# Autodesk Inventor assembly: Body
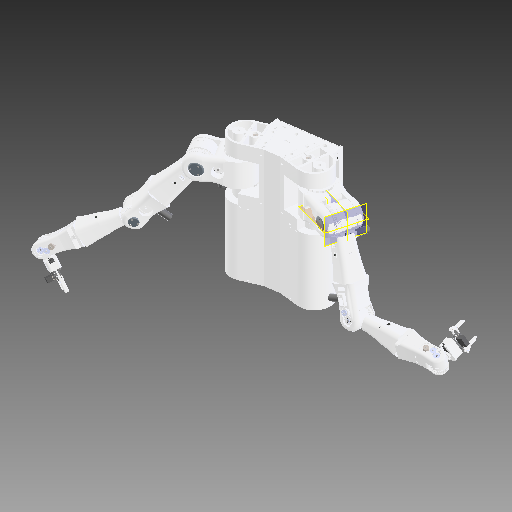
[picture p0: Inventor's stored thumbnail of the model, 512x512]
Saved by Autodesk Inventor 2017 (Build 210142000, 142)
## iProperties
Created: 2017-03-13
Part Number: Body
Document SubType Name: Assembly
Designer: zallen
Author: zallen
## Documents named in this file (4)
- C:\Users\Dell\Documents\GitHub\tr1\src\Body\Body.iam
- C:\Users\Dell\Documents\GitHub\tr1\src\Body\Chest Assembly\Chest Assembly.iam
- C:\Users\Dell\Documents\GitHub\tr1\src\Body\Arm Assembly\Arm Assembly, Right.iam
- C:\Users\Dell\Documents\GitHub\tr1\src\Body\Arm Assembly\Arm Assembly, Left.iam
## Components (3 placed, 3 different names)
1. Chest Assembly:1 [sub-assembly] — Mate:15, Mate:16, Flush:1, Mate:17, Flush:2, Mate:18
2. Arm Assembly, Right:1 [sub-assembly] — Mate:15, Mate:16, Flush:1
3. Arm Assembly, Left:1 [sub-assembly] — Mate:17, Flush:2, Mate:18
## Relationships (6: Mate 4, Flush 2)
- Mate:15: Chest Assembly:1 ↔ Arm Assembly, Right:1
- Mate:16: Chest Assembly:1 ↔ Arm Assembly, Right:1
- Flush:1: Chest Assembly:1 ↔ Arm Assembly, Right:1
- Mate:17: Chest Assembly:1 ↔ Arm Assembly, Left:1
- Flush:2: Chest Assembly:1 ↔ Arm Assembly, Left:1
- Mate:18: Chest Assembly:1 ↔ Arm Assembly, Left:1
